# Autodesk Inventor assembly: fixed_side_bk-25_
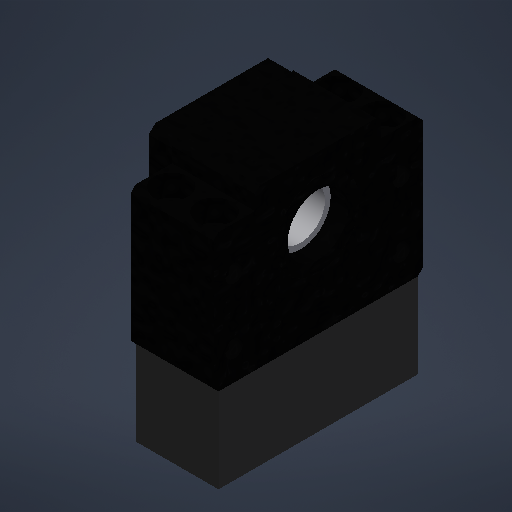
[picture p0: Inventor's stored thumbnail of the model, 512x512]
Saved by Autodesk Inventor 2025 (Build 290162000, 162)
## iProperties
Company: TraceParts S.A.
Created: 2020-01-23
Part Number: fixed_side_bk-25_
Checked By: TraceParts S.A.
Catalog Web Link: www.traceparts.com
Document SubType Name: Assembly
Designer: TraceParts
REFERENCE: BK-25
DESIGN: Fixed Side BK-25
SUPPLIER: TBI MOTION TECHNOLOGY CO., LTD.
TraceParts.PartNumber: 33-06082019-054425
TraceParts.PartTitle: Fixed Side / BK Series, Square Type
TraceParts.InstanceId: 33-06082019-05442518UKQ0UP919HIQU3JV3PWQFAD
TraceParts.PartStatus: Published
TraceParts.PartVersion: 1.0.8
TRACEPARTS: TRACEPARTS
TraceParts.PartLanguage: en
TraceParts.ClassPath: TBI_MOTION:33-06082019-054425
Author: TraceParts
## Documents named in this file (4)
- D:\UNAL\2024-1S\APM\Digital Factory\Linear Guides & Ball Screws\fixed_side_bk-25_.iam
- D:\UNAL\2024-1S\APM\Digital Factory\Linear Guides & Ball Screws\fixed_side_bk-25__01.ipt
- D:\UNAL\2024-1S\APM\Digital Factory\Linear Guides & Ball Screws\fixed_side_bk-25__02.ipt
- D:\UNAL\2024-1S\APM\Digital Factory\Packaging Machine\BaseBallScrewSupport.ipt
## Components (3 placed, 3 different names)
1. fixed_side_bk-25__01:1 — Flush:1
2. fixed_side_bk-25__02:1
3. BaseBallScrewSupport:1 — Flush:1
## Relationships (1: Flush 1)
- Flush:1: fixed_side_bk-25__01:1 ↔ BaseBallScrewSupport:1
